# Autodesk Inventor assembly: unterArm
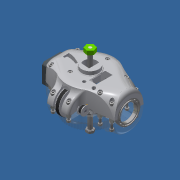
[picture p0: Inventor's stored thumbnail of the model, 180x180]
Saved by Autodesk Inventor 2016 (Build 200138000, 138)
## iProperties
Created: 2015-08-25
Part Number: unterArm
Material: Generisch
Document SubType Name: Assembly
Designer: 4ndreas
Mass: 1396.57 g
Surface Area: 1982.01 cm^2
Volume: 701.093 cm^3
Density: 1.99199 g/cm^3
Parent: R3
Author: 4ndreas
## Documents named in this file (30)
- C:\Users\4ndreas\Documents\github\Mantis-Robot-Arm\MantisRobotArm\Workspace\_assemblys\Forearm.iam
- C:\Users\4ndreas\Documents\github\Mantis-Robot-Arm\MantisRobotArm\Workspace\_assemblys\forearm\Konstruktions-Assistent\Übertragung des Zahnriemens1.iam
- C:\Users\4ndreas\Documents\github\Mantis-Robot-Arm\MantisRobotArm\Workspace\_assemblys\forearm\Konstruktions-Assistent\Übertragung des Zahnriemens2.iam
- C:\Users\4ndreas\Documents\github\Mantis-Robot-Arm\MantisRobotArm\Workspace\_motors\Nema17_60.ipt
- C:\Users\4ndreas\Documents\github\Mantis-Robot-Arm\MantisRobotArm\Workspace\_printed parts\unterArmSegment_A.ipt
- C:\Users\4ndreas\Documents\github\Mantis-Robot-Arm\MantisRobotArm\Workspace\_printed parts\unterArmSegment_B.ipt
- C:\Users\4ndreas\Documents\github\Mantis-Robot-Arm\MantisRobotArm\Libraries\Content Center Files\de-DE\DIN BEARING(1)\DIN 625 SKF - SKF 61807.ipt
- C:\Users\4ndreas\Documents\github\Mantis-Robot-Arm\MantisRobotArm\Workspace\_assemblys\forearm\Konstruktions-Assistent\Welle1.iam
- C:\Users\4ndreas\Documents\github\Mantis-Robot-Arm\MantisRobotArm\Libraries\Content Center Files\de-DE\DIN BEARING(1)\DIN 625 SKF - SKF 626.ipt
- C:\Users\4ndreas\Documents\github\Mantis-Robot-Arm\MantisRobotArm\Workspace\_metal parts\Synchrone Riemenscheibe16.ipt
- C:\Users\4ndreas\Documents\github\Mantis-Robot-Arm\MantisRobotArm\Workspace\_standard Parts\DIN 625 T1 - 619_6 - 6 x 11 x 5.ipt
- C:\Users\4ndreas\Documents\github\Mantis-Robot-Arm\MantisRobotArm\Workspace\_assemblys\forearm\Konstruktions-Assistent\Welle2.iam
- C:\Users\4ndreas\Documents\github\Mantis-Robot-Arm\MantisRobotArm\Libraries\Content Center Files\de-DE\DIN 931-1\DIN 931-1 - M8 x 55.ipt
- C:\Users\4ndreas\Documents\github\Mantis-Robot-Arm\MantisRobotArm\Workspace\_printed parts\Synchrone Riemenscheibe_60z_2.ipt
- C:\Users\4ndreas\Documents\github\Mantis-Robot-Arm\MantisRobotArm\Workspace\_encoder\EncoderMagnet.ipt
- C:\Users\4ndreas\Documents\github\Mantis-Robot-Arm\MantisRobotArm\Workspace\_printed parts\magHexMount.ipt
- C:\Users\4ndreas\Documents\github\Mantis-Robot-Arm\MantisRobotArm\Libraries\Content Center Files\de-DE\DIN 985\DIN 985 - M8.ipt
- C:\Users\4ndreas\Documents\github\Mantis-Robot-Arm\MantisRobotArm\Libraries\Content Center Files\de-DE\DIN 912\DIN 912 - M4 x 0,7 x 30 x 20.ipt
- C:\Users\4ndreas\Documents\github\Mantis-Robot-Arm\MantisRobotArm\Workspace\_standard Parts\Distanzhuelse_M4x20mm.ipt
- C:\Users\4ndreas\Documents\github\Mantis-Robot-Arm\MantisRobotArm\Libraries\Content Center Files\de-DE\DIN 913\DIN 913 - M3 x 3.ipt
- C:\Users\4ndreas\Documents\github\Mantis-Robot-Arm\MantisRobotArm\Libraries\Content Center Files\de-DE\DIN 913\DIN 913 - M3 x 8.ipt
- C:\Users\4ndreas\Documents\github\Mantis-Robot-Arm\MantisRobotArm\Workspace\_standard Parts\Distanzhuelse_M3x5mm.ipt
- C:\Users\4ndreas\Documents\github\Mantis-Robot-Arm\MantisRobotArm\Workspace\_printed parts\rotSpanner.ipt
- C:\Users\4ndreas\Documents\github\Mantis-Robot-Arm\MantisRobotArm\Libraries\Content Center Files\de-DE\DIN 912\DIN 912 - M4 x 0,7 x 16 x 14,25.ipt
- C:\Users\4ndreas\Documents\github\Mantis-Robot-Arm\MantisRobotArm\Libraries\Content Center Files\de-DE\DIN 912\DIN 912 - M4 x 0,7 x 12 x 10,25.ipt
- C:\Users\4ndreas\Documents\github\Mantis-Robot-Arm\MantisRobotArm\Libraries\Content Center Files\de-DE\DIN 912\DIN 912 - M4 x 0,7 x 25 x 23,25.ipt
- C:\Users\4ndreas\Documents\github\Mantis-Robot-Arm\MantisRobotArm\Libraries\Content Center Files\de-DE\DIN 912\DIN 912 - M3 x 0,5 x 20 x 18,75.ipt
- C:\Users\4ndreas\Documents\github\Mantis-Robot-Arm\MantisRobotArm\Libraries\Content Center Files\de-DE\DIN 985\DIN 985 - M3.ipt
- C:\Users\4ndreas\Documents\github\Mantis-Robot-Arm\MantisRobotArm\Workspace\_encoder\encoderR1_mini.ipt
- C:\Users\4ndreas\Documents\github\Mantis-Robot-Arm\MantisRobotArm\Libraries\Content Center Files\de-DE\ISO 7380-1\ISO 7380-1 - M3 x 6.ipt
## Components (76 placed, 27 different names)
1. unterArmSegment_A:1 — Passend:12, Passend:28, Passend:30, Fluchtend:1, Passend:36, Passend:41, Passend:42, Passend:100, Passend:103, Passend:106, Passend:107, Passend:47, Passend:119, Passend:130, Passend:131, Passend:136, Passend:137, Passend:159, Passend:160, Passend:161, Passend:162, Passend:163, Passend:164, Passend:165, Passend:166, Passend:167, Passend:168, Passend:169, Passend:171, Passend:172, Passend:173, Passend:174, Passend:187, Passend:188, Passend:196, Passend:197, Passend:198, Passend:199, Passend:200, Passend:201, Passend:51, Winkel:4, Passend:203, Passend:205, Passend:208, Passend:209
2. Nema17_60:1 — Fluchtend:2, Passend:32, Passend:33, Passend:39, Passend:41, Passend:42, Winkel:3
3. Übertragung des Zahnriemens:1 [sub-assembly] — Passend:27, Passend:40, Passend:112
4. Übertragung des Zahnriemens:2 [sub-assembly] — Passend:9, Passend:10, Passend:38
5. DIN 625 SKF SKF 61807:1 — Passend:9, Passend:199
6. DIN 625 SKF SKF 61807:2 — Passend:10, Passend:36
7. unterArmSegment_B:1 — Passend:12, Passend:28, Fluchtend:1, Passend:49, Passend:52, Passend:57, Passend:59, Passend:61, Passend:62, Passend:63, Passend:64, Passend:65, Passend:66, Passend:96, Passend:97, Passend:98, Passend:99, Passend:101, Passend:102, Passend:108, Winkel:3, Passend:123, Passend:124, Passend:125, Passend:140, Passend:141, Passend:142, Passend:143, Passend:191, Passend:192, Passend:195
8. Welle:1 [sub-assembly] — Passend:16, Passend:17, Passend:27, Passend:37, Passend:109, Passend:129, Tangential:1, Tangential:2, Tangential:3
9. DIN 625 SKF SKF 626:2 — Passend:16, Passend:30
10. DIN 625 SKF SKF 626:1 — Passend:17, Passend:51, Passend:110
11. Synchrone Riemenscheibe1:1 — Passend:37, Passend:38, Passend:129, Passend:144, Passend:145
12. Synchrone Riemenscheibe1:2 — Passend:39, Passend:40, Passend:146, Passend:147
13. DIN 625 - T1 619/6 - 6 x 15 x 5:1 — Passend:47, Passend:156, Fluchtend:10, Passend:204, Passend:206
14. DIN 625 - T1 619/6 - 6 x 15 x 5:2 — Passend:49, Passend:152, Fluchtend:6, Passend:207
15. DIN 625 - T1 619/6 - 6 x 15 x 5:3 — Passend:52, Passend:53, Passend:54, Fluchtend:7, Passend:153
16. DIN 625 - T1 619/6 - 6 x 15 x 5:4 — Passend:55, Passend:56, Passend:155, Fluchtend:9
17. Welle:2 [sub-assembly] — Passend:53, Passend:54, Passend:207
18. Welle:3 [sub-assembly] — Passend:55, Passend:56, Passend:204, Passend:206
19. DIN 912 - ersetzt durch DIN EN ISO 4762 M4 x 16:6 — Passend:57, Passend:59, Passend:182
20. DIN 912 - ersetzt durch DIN EN ISO 4762 M4 x 16:2 — Passend:61, Passend:64, Passend:180
21. DIN 912 - ersetzt durch DIN EN ISO 4762 M4 x 16:1 — Passend:62, Passend:63, Passend:177
22. DIN 912 - ersetzt durch DIN EN ISO 4762 M4 x 16:5 — Passend:65, Passend:66, Passend:181
23. DIN 912 - ersetzt durch DIN EN ISO 4762 M4 x 12:2 — Passend:96, Passend:98
24. DIN 912 - ersetzt durch DIN EN ISO 4762 M4 x 12:1 — Passend:97, Passend:99
25. DIN 912 - ersetzt durch DIN EN ISO 4762 M4 x 16:4 — Passend:119, Passend:123, Passend:178
26. DIN 912 - ersetzt durch DIN EN ISO 4762 M4 x 16:3 — Passend:124, Passend:125
27. DIN 931-1 - ersetzt durch DIN EN 24014 M8 x 55:1 — Passend:100, Passend:103, Passend:104, Passend:116, Passend:117, Passend:118
28. DIN 931-1 - ersetzt durch DIN EN 24014 M8 x 55:2 — Passend:101, Passend:102, Passend:105
29. DIN 985 - ersetzt durch DIN EN ISO 10511 M8:1 — Passend:104, Fluchtend:3, Passend:106, Passend:107
30. DIN 985 - ersetzt durch DIN EN ISO 10511 M8:2 — Passend:105, Fluchtend:3, Passend:108
31. Synchrone Riemenscheibe2:1 — Passend:109, Passend:110, Passend:149, Passend:150, Passend:151
32. EncoderMagnet:1 — Passend:114, Passend:115
33. magHexMount:1 — Passend:114, Passend:115, Passend:116, Passend:117, Passend:118
34. Distanzhuelse_M4x20mm:1 — Passend:131, Fluchtend:15, Fluchtend:18
35. Distanzhuelse_M4x20mm:2 — Passend:130, Fluchtend:19, Fluchtend:23
36. DIN 912 - ersetzt durch DIN EN ISO 4762 M4 x 30:1 — Passend:137
37. DIN 912 - ersetzt durch DIN EN ISO 4762 M4 x 30:2 — Passend:136
38. DIN 912 - ersetzt durch DIN EN ISO 4762 M4 x 30:3 — Passend:140, Passend:142
39. DIN 912 - ersetzt durch DIN EN ISO 4762 M4 x 30:4 — Passend:141, Passend:143
40. DIN 913 M3 x 3:1 — Tangential:2, Passend:145
41. DIN 913 M3 x 3:2 — Tangential:1, Passend:144
42. DIN 913 M3 x 3:3 — Passend:147
43. DIN 913 M3 x 3:4 — Passend:146
44. DIN 913 M3 x 8:1 — Passend:148, Passend:149, Tangential:3
45. Distanzhuelse_M3x5mm:1 — Passend:148, Passend:150, Passend:151
46. rotSpanner:1 — Fluchtend:7, Passend:153, Fluchtend:8, Fluchtend:12, Passend:190
47. rotSpanner:2 — Passend:152, Fluchtend:6, Fluchtend:8, Passend:189, Passend:208
48. rotSpanner:3 — Passend:155, Fluchtend:9, Fluchtend:11, Passend:194
49. rotSpanner:4 — Passend:156, Fluchtend:10, Fluchtend:11, Fluchtend:12, Passend:193, Passend:205
50. DIN 912 - ersetzt durch DIN EN ISO 4762 M4 x 12:3 — Passend:160, Passend:161, Passend:175
51. DIN 912 - ersetzt durch DIN EN ISO 4762 M4 x 12:4 — Passend:159, Passend:162, Passend:176
52. DIN 912 - ersetzt durch DIN EN ISO 4762 M4 x 16:7 — Passend:163, Passend:165
53. DIN 912 - ersetzt durch DIN EN ISO 4762 M4 x 16:8 — Passend:164, Passend:166, Passend:179
54. DIN 912 - ersetzt durch DIN EN ISO 4762 M4 x 25:1 — Passend:168, Passend:169
55. DIN 912 - ersetzt durch DIN EN ISO 4762 M4 x 25:2 — Passend:167, Passend:198
56. DIN 912 - ersetzt durch DIN EN ISO 4762 M4 x 25:4 — Passend:172, Passend:174
57. DIN 912 - ersetzt durch DIN EN ISO 4762 M4 x 25:3 — Passend:171, Passend:173
58. Distanzhuelse_M4x20mm:3 — Passend:179, Fluchtend:17, Fluchtend:20
59. Distanzhuelse_M4x20mm:4 — Passend:177, Fluchtend:13, Fluchtend:14, Fluchtend:15, Fluchtend:16
60. Distanzhuelse_M4x20mm:5 — Passend:175, Fluchtend:14, Passend:200, Passend:209
61. Distanzhuelse_M4x20mm:6 — Passend:178, Fluchtend:16, Fluchtend:17
62. Distanzhuelse_M4x20mm:7 — Passend:176, Fluchtend:13, Passend:201
63. Distanzhuelse_M4x20mm:8 — Passend:180, Fluchtend:20, Fluchtend:23
64. Distanzhuelse_M4x20mm:9 — Passend:181, Fluchtend:19
65. Distanzhuelse_M4x20mm:10 — Passend:182, Fluchtend:18
66. DIN 912 - ersetzt durch DIN EN ISO 4762 M3 x 20:1 — Passend:183, Passend:187, Passend:190
67. DIN 985 - ersetzt durch DIN EN ISO 10511 M3:1 — Passend:183, Fluchtend:21, Passend:196, Passend:197
68. DIN 912 - ersetzt durch DIN EN ISO 4762 M3 x 20:2 — Passend:192, Passend:194
69. DIN 985 - ersetzt durch DIN EN ISO 10511 M3:2 — Fluchtend:22
70. DIN 912 - ersetzt durch DIN EN ISO 4762 M3 x 20:3 — Passend:191, Passend:193
71. DIN 985 - ersetzt durch DIN EN ISO 10511 M3:3 — Passend:195, Fluchtend:22
72. DIN 912 - ersetzt durch DIN EN ISO 4762 M3 x 20:4 — Passend:188, Passend:189
73. DIN 985 - ersetzt durch DIN EN ISO 10511 M3:4 — Fluchtend:21
74. encoderR1_mini:1 — Passend:202, Winkel:4, Passend:203, Einfügen:1, Einfügen:3
75. ISO 7380-1 M3 x 6:1 — Einfügen:1
76. ISO 7380-1 M3 x 6:3 — Einfügen:3
## Relationships (157: Mate 129, Flush 21, Tangent 3, Angle 2, Insert 2)
- Passend:9 [Mate]: Übertragung des Zahnriemens:2 ↔ DIN 625 SKF SKF 61807:1
- Passend:10 [Mate]: Übertragung des Zahnriemens:2 ↔ DIN 625 SKF SKF 61807:2
- Passend:12 [Mate]: unterArmSegment_A:1 ↔ unterArmSegment_B:1
- Passend:16 [Mate]: Welle:1 ↔ DIN 625 SKF SKF 626:2
- Passend:17 [Mate]: Welle:1 ↔ DIN 625 SKF SKF 626:1
- Passend:27 [Mate]: Übertragung des Zahnriemens:1 ↔ Welle:1
- Passend:28 [Mate]: unterArmSegment_A:1 ↔ unterArmSegment_B:1
- Passend:30 [Mate]: unterArmSegment_A:1 ↔ DIN 625 SKF SKF 626:2
- Fluchtend:1 [Flush]: unterArmSegment_A:1 ↔ unterArmSegment_B:1
- Fluchtend:2 [Flush]: Nema17_60:1
- Passend:32 [Mate]: Nema17_60:1
- Passend:33 [Mate]: Nema17_60:1
- Passend:36 [Mate]: unterArmSegment_A:1 ↔ DIN 625 SKF SKF 61807:2
- Passend:37 [Mate]: Welle:1 ↔ Synchrone Riemenscheibe1:1
- Passend:38 [Mate] (0.25 mm): Übertragung des Zahnriemens:2 ↔ Synchrone Riemenscheibe1:1
- Passend:39 [Mate]: Nema17_60:1 ↔ Synchrone Riemenscheibe1:2
- Passend:40 [Mate] (0.25 mm): Übertragung des Zahnriemens:1 ↔ Synchrone Riemenscheibe1:2
- Passend:41 [Mate]: unterArmSegment_A:1 ↔ Nema17_60:1
- Passend:42 [Mate]: unterArmSegment_A:1 ↔ Nema17_60:1
- Passend:47 [Mate]: unterArmSegment_A:1 ↔ DIN 625 - T1 619/6 - 6 x 15 x 5:1
- Passend:49 [Mate]: unterArmSegment_B:1 ↔ DIN 625 - T1 619/6 - 6 x 15 x 5:2
- Passend:51 [Mate]: unterArmSegment_A:1 ↔ DIN 625 SKF SKF 626:1
- Passend:52 [Mate]: unterArmSegment_B:1 ↔ DIN 625 - T1 619/6 - 6 x 15 x 5:3
- Passend:53 [Mate]: DIN 625 - T1 619/6 - 6 x 15 x 5:3 ↔ Welle:2
- Passend:54 [Mate]: DIN 625 - T1 619/6 - 6 x 15 x 5:3 ↔ Welle:2
- Passend:55 [Mate]: DIN 625 - T1 619/6 - 6 x 15 x 5:4 ↔ Welle:3
- Passend:56 [Mate]: DIN 625 - T1 619/6 - 6 x 15 x 5:4 ↔ Welle:3
- Passend:57 [Mate]: unterArmSegment_B:1 ↔ DIN 912 - ersetzt durch DIN EN ISO 4762 M4 x 16:6
- Passend:59 [Mate]: unterArmSegment_B:1 ↔ DIN 912 - ersetzt durch DIN EN ISO 4762 M4 x 16:6
- Passend:61 [Mate]: unterArmSegment_B:1 ↔ DIN 912 - ersetzt durch DIN EN ISO 4762 M4 x 16:2
- Passend:62 [Mate]: unterArmSegment_B:1 ↔ DIN 912 - ersetzt durch DIN EN ISO 4762 M4 x 16:1
- Passend:63 [Mate]: unterArmSegment_B:1 ↔ DIN 912 - ersetzt durch DIN EN ISO 4762 M4 x 16:1
- Passend:64 [Mate]: unterArmSegment_B:1 ↔ DIN 912 - ersetzt durch DIN EN ISO 4762 M4 x 16:2
- Passend:65 [Mate]: unterArmSegment_B:1 ↔ DIN 912 - ersetzt durch DIN EN ISO 4762 M4 x 16:5
- Passend:66 [Mate]: unterArmSegment_B:1 ↔ DIN 912 - ersetzt durch DIN EN ISO 4762 M4 x 16:5
- Passend:96 [Mate]: unterArmSegment_B:1 ↔ DIN 912 - ersetzt durch DIN EN ISO 4762 M4 x 12:2
- Passend:97 [Mate]: unterArmSegment_B:1 ↔ DIN 912 - ersetzt durch DIN EN ISO 4762 M4 x 12:1
- Passend:98 [Mate]: unterArmSegment_B:1 ↔ DIN 912 - ersetzt durch DIN EN ISO 4762 M4 x 12:2
- Passend:99 [Mate]: unterArmSegment_B:1 ↔ DIN 912 - ersetzt durch DIN EN ISO 4762 M4 x 12:1
- Passend:100 [Mate]: unterArmSegment_A:1 ↔ DIN 931-1 - ersetzt durch DIN EN 24014 M8 x 55:1
- Passend:101 [Mate]: unterArmSegment_B:1 ↔ DIN 931-1 - ersetzt durch DIN EN 24014 M8 x 55:2
- Passend:102 [Mate] (28 mm): unterArmSegment_B:1 ↔ DIN 931-1 - ersetzt durch DIN EN 24014 M8 x 55:2
- Passend:103 [Mate] (29 mm): unterArmSegment_A:1 ↔ DIN 931-1 - ersetzt durch DIN EN 24014 M8 x 55:1
- Passend:104 [Mate]: DIN 931-1 - ersetzt durch DIN EN 24014 M8 x 55:1 ↔ DIN 985 - ersetzt durch DIN EN ISO 10511 M8:1
- Passend:105 [Mate]: DIN 931-1 - ersetzt durch DIN EN 24014 M8 x 55:2 ↔ DIN 985 - ersetzt durch DIN EN ISO 10511 M8:2
- Fluchtend:3 [Flush]: DIN 985 - ersetzt durch DIN EN ISO 10511 M8:1 ↔ DIN 985 - ersetzt durch DIN EN ISO 10511 M8:2
- Passend:106 [Mate]: unterArmSegment_A:1 ↔ DIN 985 - ersetzt durch DIN EN ISO 10511 M8:1
- Passend:107 [Mate]: unterArmSegment_A:1 ↔ DIN 985 - ersetzt durch DIN EN ISO 10511 M8:1
- Passend:108 [Mate]: unterArmSegment_B:1 ↔ DIN 985 - ersetzt durch DIN EN ISO 10511 M8:2
- Passend:109 [Mate]: Welle:1 ↔ Synchrone Riemenscheibe2:1
- Passend:110 [Mate]: DIN 625 SKF SKF 626:1 ↔ Synchrone Riemenscheibe2:1
- Passend:112 [Mate]: Übertragung des Zahnriemens:1
- Winkel:3 [Angle] (0 deg): Nema17_60:1 ↔ unterArmSegment_B:1
- Passend:114 [Mate]: EncoderMagnet:1 ↔ magHexMount:1
- Passend:115 [Mate]: EncoderMagnet:1 ↔ magHexMount:1
- Passend:116 [Mate]: DIN 931-1 - ersetzt durch DIN EN 24014 M8 x 55:1 ↔ magHexMount:1
- Passend:117 [Mate]: DIN 931-1 - ersetzt durch DIN EN 24014 M8 x 55:1 ↔ magHexMount:1
- Passend:118 [Mate]: DIN 931-1 - ersetzt durch DIN EN 24014 M8 x 55:1 ↔ magHexMount:1
- Passend:119 [Mate]: unterArmSegment_A:1 ↔ DIN 912 - ersetzt durch DIN EN ISO 4762 M4 x 16:4
- Passend:123 [Mate]: unterArmSegment_B:1 ↔ DIN 912 - ersetzt durch DIN EN ISO 4762 M4 x 16:4
- Passend:124 [Mate]: unterArmSegment_B:1 ↔ DIN 912 - ersetzt durch DIN EN ISO 4762 M4 x 16:3
- Passend:125 [Mate]: unterArmSegment_B:1 ↔ DIN 912 - ersetzt durch DIN EN ISO 4762 M4 x 16:3
- Passend:129 [Mate]: Welle:1 ↔ Synchrone Riemenscheibe1:1
- Passend:130 [Mate]: unterArmSegment_A:1 ↔ Distanzhuelse_M4x20mm:2
- Passend:131 [Mate]: unterArmSegment_A:1 ↔ Distanzhuelse_M4x20mm:1
- Passend:136 [Mate]: unterArmSegment_A:1 ↔ DIN 912 - ersetzt durch DIN EN ISO 4762 M4 x 30:2
- Passend:137 [Mate]: unterArmSegment_A:1 ↔ DIN 912 - ersetzt durch DIN EN ISO 4762 M4 x 30:1
- Passend:140 [Mate]: unterArmSegment_B:1 ↔ DIN 912 - ersetzt durch DIN EN ISO 4762 M4 x 30:3
- Passend:141 [Mate]: unterArmSegment_B:1 ↔ DIN 912 - ersetzt durch DIN EN ISO 4762 M4 x 30:4
- Passend:142 [Mate]: unterArmSegment_B:1 ↔ DIN 912 - ersetzt durch DIN EN ISO 4762 M4 x 30:3
- Passend:143 [Mate]: unterArmSegment_B:1 ↔ DIN 912 - ersetzt durch DIN EN ISO 4762 M4 x 30:4
- Tangential:1: Welle:1 ↔ DIN 913 M3 x 3:2
- Tangential:2: Welle:1 ↔ DIN 913 M3 x 3:1
- Passend:144 [Mate]: Synchrone Riemenscheibe1:1 ↔ DIN 913 M3 x 3:2
- Passend:145 [Mate]: Synchrone Riemenscheibe1:1 ↔ DIN 913 M3 x 3:1
- Passend:146 [Mate]: Synchrone Riemenscheibe1:2 ↔ DIN 913 M3 x 3:4
- Passend:147 [Mate]: Synchrone Riemenscheibe1:2 ↔ DIN 913 M3 x 3:3
- Passend:148 [Mate]: DIN 913 M3 x 8:1 ↔ Distanzhuelse_M3x5mm:1
- Passend:149 [Mate]: Synchrone Riemenscheibe2:1 ↔ DIN 913 M3 x 8:1
- Passend:150 [Mate]: Synchrone Riemenscheibe2:1 ↔ Distanzhuelse_M3x5mm:1
- Passend:151 [Mate]: Synchrone Riemenscheibe2:1 ↔ Distanzhuelse_M3x5mm:1
- Tangential:3: Welle:1 ↔ DIN 913 M3 x 8:1
- Passend:152 [Mate]: DIN 625 - T1 619/6 - 6 x 15 x 5:2 ↔ rotSpanner:2
- Fluchtend:6 [Flush]: DIN 625 - T1 619/6 - 6 x 15 x 5:2 ↔ rotSpanner:2
- Fluchtend:7 [Flush]: DIN 625 - T1 619/6 - 6 x 15 x 5:3 ↔ rotSpanner:1
- Passend:153 [Mate]: DIN 625 - T1 619/6 - 6 x 15 x 5:3 ↔ rotSpanner:1
- Fluchtend:8 [Flush]: rotSpanner:1 ↔ rotSpanner:2
- Passend:155 [Mate]: DIN 625 - T1 619/6 - 6 x 15 x 5:4 ↔ rotSpanner:3
- Fluchtend:9 [Flush]: DIN 625 - T1 619/6 - 6 x 15 x 5:4 ↔ rotSpanner:3
- Passend:156 [Mate]: DIN 625 - T1 619/6 - 6 x 15 x 5:1 ↔ rotSpanner:4
- Fluchtend:10 [Flush]: DIN 625 - T1 619/6 - 6 x 15 x 5:1 ↔ rotSpanner:4
- Fluchtend:11 [Flush]: rotSpanner:3 ↔ rotSpanner:4
- Fluchtend:12 [Flush]: rotSpanner:1 ↔ rotSpanner:4
- Passend:159 [Mate]: unterArmSegment_A:1 ↔ DIN 912 - ersetzt durch DIN EN ISO 4762 M4 x 12:4
- Passend:160 [Mate]: unterArmSegment_A:1 ↔ DIN 912 - ersetzt durch DIN EN ISO 4762 M4 x 12:3
- Passend:161 [Mate]: unterArmSegment_A:1 ↔ DIN 912 - ersetzt durch DIN EN ISO 4762 M4 x 12:3
- Passend:162 [Mate]: unterArmSegment_A:1 ↔ DIN 912 - ersetzt durch DIN EN ISO 4762 M4 x 12:4
- Passend:163 [Mate]: unterArmSegment_A:1 ↔ DIN 912 - ersetzt durch DIN EN ISO 4762 M4 x 16:7
- Passend:164 [Mate]: unterArmSegment_A:1 ↔ DIN 912 - ersetzt durch DIN EN ISO 4762 M4 x 16:8
- Passend:165 [Mate]: unterArmSegment_A:1 ↔ DIN 912 - ersetzt durch DIN EN ISO 4762 M4 x 16:7
- Passend:166 [Mate]: unterArmSegment_A:1 ↔ DIN 912 - ersetzt durch DIN EN ISO 4762 M4 x 16:8
- Passend:167 [Mate]: unterArmSegment_A:1 ↔ DIN 912 - ersetzt durch DIN EN ISO 4762 M4 x 25:2
- Passend:168 [Mate]: unterArmSegment_A:1 ↔ DIN 912 - ersetzt durch DIN EN ISO 4762 M4 x 25:1
- Passend:169 [Mate]: unterArmSegment_A:1 ↔ DIN 912 - ersetzt durch DIN EN ISO 4762 M4 x 25:1
- Passend:171 [Mate]: unterArmSegment_A:1 ↔ DIN 912 - ersetzt durch DIN EN ISO 4762 M4 x 25:3
- Passend:172 [Mate]: unterArmSegment_A:1 ↔ DIN 912 - ersetzt durch DIN EN ISO 4762 M4 x 25:4
- Passend:173 [Mate]: unterArmSegment_A:1 ↔ DIN 912 - ersetzt durch DIN EN ISO 4762 M4 x 25:3
- Passend:174 [Mate]: unterArmSegment_A:1 ↔ DIN 912 - ersetzt durch DIN EN ISO 4762 M4 x 25:4
- Passend:175 [Mate]: DIN 912 - ersetzt durch DIN EN ISO 4762 M4 x 12:3 ↔ Distanzhuelse_M4x20mm:5
- Passend:176 [Mate]: DIN 912 - ersetzt durch DIN EN ISO 4762 M4 x 12:4 ↔ Distanzhuelse_M4x20mm:7
- Passend:177 [Mate]: DIN 912 - ersetzt durch DIN EN ISO 4762 M4 x 16:1 ↔ Distanzhuelse_M4x20mm:4
- Passend:178 [Mate]: DIN 912 - ersetzt durch DIN EN ISO 4762 M4 x 16:4 ↔ Distanzhuelse_M4x20mm:6
- Passend:179 [Mate]: DIN 912 - ersetzt durch DIN EN ISO 4762 M4 x 16:8 ↔ Distanzhuelse_M4x20mm:3
- Fluchtend:13 [Flush]: Distanzhuelse_M4x20mm:4 ↔ Distanzhuelse_M4x20mm:7
- Fluchtend:14 [Flush]: Distanzhuelse_M4x20mm:4 ↔ Distanzhuelse_M4x20mm:5
- Fluchtend:15 [Flush]: Distanzhuelse_M4x20mm:1 ↔ Distanzhuelse_M4x20mm:4
- Fluchtend:16 [Flush]: Distanzhuelse_M4x20mm:4 ↔ Distanzhuelse_M4x20mm:6
- Fluchtend:17 [Flush]: Distanzhuelse_M4x20mm:3 ↔ Distanzhuelse_M4x20mm:6
- Passend:180 [Mate]: DIN 912 - ersetzt durch DIN EN ISO 4762 M4 x 16:2 ↔ Distanzhuelse_M4x20mm:8
- Passend:181 [Mate]: DIN 912 - ersetzt durch DIN EN ISO 4762 M4 x 16:5 ↔ Distanzhuelse_M4x20mm:9
- Passend:182 [Mate]: DIN 912 - ersetzt durch DIN EN ISO 4762 M4 x 16:6 ↔ Distanzhuelse_M4x20mm:10
- Fluchtend:18 [Flush]: Distanzhuelse_M4x20mm:1 ↔ Distanzhuelse_M4x20mm:10
- Fluchtend:19 [Flush]: Distanzhuelse_M4x20mm:2 ↔ Distanzhuelse_M4x20mm:9
- Fluchtend:20 [Flush]: Distanzhuelse_M4x20mm:3 ↔ Distanzhuelse_M4x20mm:8
- Passend:183 [Mate]: DIN 912 - ersetzt durch DIN EN ISO 4762 M3 x 20:1 ↔ DIN 985 - ersetzt durch DIN EN ISO 10511 M3:1
- [Mate]: DIN 912 - ersetzt durch DIN EN ISO 4762 M3 x 20:2 ↔ DIN 985 - ersetzt durch DIN EN ISO 10511 M3:2
- [Mate]: DIN 912 - ersetzt durch DIN EN ISO 4762 M3 x 20:3 ↔ DIN 985 - ersetzt durch DIN EN ISO 10511 M3:3
- [Mate]: DIN 912 - ersetzt durch DIN EN ISO 4762 M3 x 20:4 ↔ DIN 985 - ersetzt durch DIN EN ISO 10511 M3:4
- Passend:187 [Mate]: unterArmSegment_A:1 ↔ DIN 912 - ersetzt durch DIN EN ISO 4762 M3 x 20:1
- Passend:188 [Mate]: unterArmSegment_A:1 ↔ DIN 912 - ersetzt durch DIN EN ISO 4762 M3 x 20:4
- Passend:189 [Mate]: rotSpanner:2 ↔ DIN 912 - ersetzt durch DIN EN ISO 4762 M3 x 20:4
- Passend:190 [Mate]: rotSpanner:1 ↔ DIN 912 - ersetzt durch DIN EN ISO 4762 M3 x 20:1
- Fluchtend:21 [Flush]: DIN 985 - ersetzt durch DIN EN ISO 10511 M3:1 ↔ DIN 985 - ersetzt durch DIN EN ISO 10511 M3:4
- Passend:191 [Mate]: unterArmSegment_B:1 ↔ DIN 912 - ersetzt durch DIN EN ISO 4762 M3 x 20:3
- Passend:192 [Mate]: unterArmSegment_B:1 ↔ DIN 912 - ersetzt durch DIN EN ISO 4762 M3 x 20:2
- Passend:193 [Mate]: rotSpanner:4 ↔ DIN 912 - ersetzt durch DIN EN ISO 4762 M3 x 20:3
- Passend:194 [Mate]: rotSpanner:3 ↔ DIN 912 - ersetzt durch DIN EN ISO 4762 M3 x 20:2
- Passend:195 [Mate]: unterArmSegment_B:1 ↔ DIN 985 - ersetzt durch DIN EN ISO 10511 M3:3
- Fluchtend:22 [Flush]: DIN 985 - ersetzt durch DIN EN ISO 10511 M3:2 ↔ DIN 985 - ersetzt durch DIN EN ISO 10511 M3:3
- Passend:196 [Mate]: unterArmSegment_A:1 ↔ DIN 985 - ersetzt durch DIN EN ISO 10511 M3:1
- Passend:197 [Mate]: unterArmSegment_A:1 ↔ DIN 985 - ersetzt durch DIN EN ISO 10511 M3:1
- Passend:198 [Mate]: unterArmSegment_A:1 ↔ DIN 912 - ersetzt durch DIN EN ISO 4762 M4 x 25:2
- Passend:199 [Mate]: unterArmSegment_A:1 ↔ DIN 625 SKF SKF 61807:1
- Passend:200 [Mate]: unterArmSegment_A:1 ↔ Distanzhuelse_M4x20mm:5
- Passend:201 [Mate]: unterArmSegment_A:1 ↔ Distanzhuelse_M4x20mm:7
- Passend:202 [Mate]: encoderR1_mini:1
- Winkel:4 [Angle] (0 deg): unterArmSegment_A:1 ↔ encoderR1_mini:1
- Passend:203 [Mate]: unterArmSegment_A:1 ↔ encoderR1_mini:1
- Einfügen:1 [Insert]: encoderR1_mini:1 ↔ ISO 7380-1 M3 x 6:1
- Einfügen:3 [Insert]: encoderR1_mini:1 ↔ ISO 7380-1 M3 x 6:3
- Passend:204 [Mate]: DIN 625 - T1 619/6 - 6 x 15 x 5:1 ↔ Welle:3
- Passend:205 [Mate]: unterArmSegment_A:1 ↔ rotSpanner:4
- Passend:206 [Mate]: DIN 625 - T1 619/6 - 6 x 15 x 5:1 ↔ Welle:3
- Passend:207 [Mate]: DIN 625 - T1 619/6 - 6 x 15 x 5:2 ↔ Welle:2
- Passend:208 [Mate]: unterArmSegment_A:1 ↔ rotSpanner:2
- Fluchtend:23 [Flush]: Distanzhuelse_M4x20mm:2 ↔ Distanzhuelse_M4x20mm:8
- Passend:209 [Mate]: unterArmSegment_A:1 ↔ Distanzhuelse_M4x20mm:5
## Named parameters: d233_d232 = 0 mm, d234_d232 = 0 mm, d235_d232 = 0 mm
